# Autodesk Inventor assembly: Miras
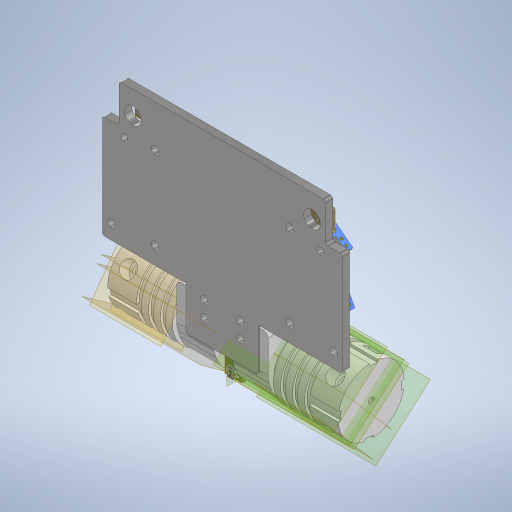
[picture p0: Inventor's stored thumbnail of the model, 512x512]
Saved by Autodesk Inventor 2023.5 (Build 275446000, 446)
## iProperties
Created: 2022-12-28
Part Number: Miras
Document SubType Name: Assembly
Designer: Kamil
Author: Kamil
## Documents named in this file (27)
- E:\PROJECTS_REPOS\Miras\mechanics\Miras.iam
- E:\PROJECTS_REPOS\Miras\mechanics\steel_2.ipt
- E:\PROJECTS_REPOS\Miras\mechanics\lead_3.ipt
- E:\PROJECTS_REPOS\Miras\mechanics\Part8.ipt
- E:\PROJECTS_REPOS\Miras\mechanics\n20 motor.ipt
- E:\PROJECTS_REPOS\Miras\mechanics\felga.ipt
- E:\PROJECTS_REPOS\Miras\mechanics\opona.ipt
- E:\PROJECTS_REPOS\Miras\mechanics\strug.ipt
- E:\PROJECTS_REPOS\Miras\mechanics\sciana.ipt
- E:\PROJECTS_REPOS\Miras\mechanics\sciana_MIR.ipt
- E:\PROJECTS_REPOS\Miras\mechanics\uchwyt na plytke.ipt
- E:\PROJECTS_REPOS\Miras\mechanics\wachlarz_1.ipt
- E:\PROJECTS_REPOS\Miras\mechanics\wachlarz_1_MIR.ipt
- E:\PROJECTS_REPOS\Miras\mechanics\Serwo_z_widelcem.iam
- E:\PROJECTS_REPOS\Miras\mechanics\widelec.ipt
- E:\PROJECTS_REPOS\Miras\mechanics\faulhaber_motor.ipt
- E:\PROJECTS_REPOS\Miras\mechanics\motors_mount_miras.ipt
- E:\PROJECTS_REPOS\Miras\mechanics\wymiar.ipt
- E:\PROJECTS_REPOS\Miras\mechanics\kolo_tetsowe.ipt
- E:\PROJECTS_REPOS\Miras\mechanics\pcb_podstawka.ipt
- E:\PROJECTS_REPOS\Miras\mechanics\plytka_stal_3mm\plytka_stal_3mm.ipt
- E:\PROJECTS_REPOS\Miras\mechanics\pokrywa_stal_3mm\pokrywa_stal_3mm.ipt
- E:\PROJECTS_REPOS\Miras\mechanics\pcb_main_miras v4.ipt
- E:\PROJECTS_REPOS\Miras\mechanics\pcb_top v5.ipt
- E:\PROJECTS_REPOS\Miras\mechanics\Weewooday I2C OLED 0.98_ 128x64.ipt
- C:\Users\kamil\Downloads\Motor\Motor.ipt
- E:\PROJECTS_REPOS\Miras\mechanics\mototrs_Mount_miras_pololu_n20.ipt
## Components (32 placed, 26 different names)
1. steel_2:1 — Mate:4, Mate:5, Flush:1
2. lead_3:1 — Mate:4, Mate:5, Flush:1, Flush:2, Flush:3, Mate:16
3. Part8:1 — Flush:2, Flush:3, Mate:11, Mate:12, Mate:13, Mate:14, Mate:15, Mate:18, Mate:55
4. n20 motor:1 — Mate:10, Mate:11, Mate:13, Mate:14, Mate:19, Mate:20, Mate:21
5. n20 motor:2 — Mate:10, Mate:12, Mate:15, Mate:16, Mate:17, Mate:22
6. felga:1 — Mate:17, Mate:18, Mate:22, Mate:24, Mate:25
7. felga:2 — Mate:19, Mate:20, Mate:21, Mate:23, Mate:26
8. opona:1 — Mate:23, Mate:26, Zestawiające:63
9. opona:2 — Mate:24, Mate:25
10. strug:1 — Mate:29, Mate:31, Zestawiające:68, Równoległe:26, Zestawiające:76, Zestawiające:78
11. sciana:1 — Mate:29, Zestawiające:74, Równoległe:27, Zestawiające:76, Równoległe:28
12. sciana_MIR:1 — Mate:31, Zestawiające:77
13. uchwyt na plytke:1 — Zestawiające:83, Zestawiające:84, Zestawiające:85, Zestawiające:87, Równoległe:30, Zestawiające:88, Zestawiające:89
14. wachlarz_1:2 — Flush:16
15. wachlarz_1_MIR:1 — Flush:16
16. widelec:1 — Mate:55, Mate:56, Mate:57
17. Serwo_z_widelcem:1 [sub-assembly] — Mate:56, Mate:57
18. faulhaber_motor:1 — Kątowe:1, Zestawiające:62, Zestawiające:72
19. faulhaber_motor:2 — Kątowe:1, Zestawiające:62, Zestawiające:63, Zestawiające:71, Zestawiające:73
20. motors_mount_miras:1 — Zestawiające:69, Zestawiające:71, Zestawiające:72, Zestawiające:73, Zestawiające:75, Kątowe:2, Zestawiające:83, Zestawiające:84, Równoległe:30
21. wymiar:1 — Zestawiające:68, Równoległe:26, Zestawiające:69
22. kolo_tetsowe:1 — Zestawiające:91, Zestawiające:93
23. kolo_tetsowe:2 — Zestawiające:90, Zestawiające:92
24. pcb_podstawka:1 — Zestawiające:79, Zestawiające:80, Zestawiające:81, Zestawiające:82
25. plytka_stal_3mm:1 — Zestawiające:74, Równoległe:27, Zestawiające:75, Zestawiające:82, Równoległe:29, Zestawiające:94, Zestawiające:95
26. pokrywa_stal_3mm:1 — Zestawiające:77, Równoległe:28, Zestawiające:78
27. pcb_main_miras v4:1 — Zestawiające:79, Zestawiające:80, Zestawiające:81, Kątowe:2, Równoległe:29, Równoległe:32
28. pcb_top v5:1 — Zestawiające:85
29. Weewooday I2C OLED 0.98_ 128x64:1 — Zestawiające:87, Zestawiające:88, Zestawiające:89
30. Motor:1 — Zestawiające:90, Równoległe:31, Zestawiające:92, Kątowe:3
31. Motor:2 — Zestawiające:91, Równoległe:31, Zestawiające:93
32. mototrs_Mount_miras_pololu_n20:1 — Zestawiające:94, Równoległe:32, Kątowe:3, Zestawiające:95
## Relationships (66: Mate 52, Flush 11, Angle 3)
- Mate:4: steel_2:1 ↔ lead_3:1
- Mate:5: steel_2:1 ↔ lead_3:1
- Flush:1: steel_2:1 ↔ lead_3:1
- Flush:2: lead_3:1 ↔ Part8:1
- Flush:3: lead_3:1 ↔ Part8:1
- Mate:10 (5 mm): n20 motor:1 ↔ n20 motor:2
- Mate:11 (2.5 mm): Part8:1 ↔ n20 motor:1
- Mate:12: Part8:1 ↔ n20 motor:2
- Mate:13: Part8:1 ↔ n20 motor:1
- Mate:14: Part8:1 ↔ n20 motor:1
- Mate:15: Part8:1 ↔ n20 motor:2
- Mate:16: lead_3:1 ↔ n20 motor:2
- Mate:17 (0.5 mm): n20 motor:2 ↔ felga:1
- Mate:18: Part8:1 ↔ felga:1
- Mate:19 (0.5 mm): n20 motor:1 ↔ felga:2
- Mate:20: n20 motor:1 ↔ felga:2
- Mate:21: n20 motor:1 ↔ felga:2
- Mate:22: n20 motor:2 ↔ felga:1
- Mate:23: felga:2 ↔ opona:1
- Mate:24: felga:1 ↔ opona:2
- Mate:25: felga:1 ↔ opona:2
- Mate:26: felga:2 ↔ opona:1
- Mate:29: strug:1 ↔ sciana:1
- Mate:31: strug:1 ↔ sciana_MIR:1
- Flush:16: wachlarz_1:2 ↔ wachlarz_1_MIR:1
- Mate:55: Part8:1 ↔ widelec:1
- Mate:56 (0.5 mm): widelec:1 ↔ Serwo_z_widelcem:1
- Mate:57: widelec:1 ↔ Serwo_z_widelcem:1
- Kątowe:1 [Angle] (180 deg): faulhaber_motor:1 ↔ faulhaber_motor:2
- Zestawiające:62 [Mate]: faulhaber_motor:1 ↔ faulhaber_motor:2
- Zestawiające:63 [Mate]: opona:1 ↔ faulhaber_motor:2
- Zestawiające:68 [Mate]: strug:1 ↔ wymiar:1
- Równoległe:26 [Flush]: strug:1 ↔ wymiar:1
- Zestawiające:69 [Mate] (-50 mm): motors_mount_miras:1 ↔ wymiar:1
- Zestawiające:71 [Mate]: faulhaber_motor:2 ↔ motors_mount_miras:1
- Zestawiające:72 [Mate]: faulhaber_motor:1 ↔ motors_mount_miras:1
- Zestawiające:73 [Mate]: faulhaber_motor:2 ↔ motors_mount_miras:1
- Zestawiające:74 [Mate]: sciana:1 ↔ plytka_stal_3mm:1
- Równoległe:27 [Flush]: sciana:1 ↔ plytka_stal_3mm:1
- Zestawiające:75 [Mate]: motors_mount_miras:1 ↔ plytka_stal_3mm:1
- Zestawiające:76 [Mate]: strug:1 ↔ sciana:1
- Zestawiające:77 [Mate]: sciana_MIR:1 ↔ pokrywa_stal_3mm:1
- Równoległe:28 [Flush]: sciana:1 ↔ pokrywa_stal_3mm:1
- Zestawiające:78 [Mate]: strug:1 ↔ pokrywa_stal_3mm:1
- Zestawiające:79 [Mate]: pcb_podstawka:1 ↔ pcb_main_miras v4:1
- Zestawiające:80 [Mate]: pcb_podstawka:1 ↔ pcb_main_miras v4:1
- Zestawiające:81 [Mate]: pcb_podstawka:1 ↔ pcb_main_miras v4:1
- Zestawiające:82 [Mate]: pcb_podstawka:1 ↔ plytka_stal_3mm:1
- Kątowe:2 [Angle] (0 deg): motors_mount_miras:1 ↔ pcb_main_miras v4:1
- Równoległe:29 [Flush] (-2 mm): plytka_stal_3mm:1 ↔ pcb_main_miras v4:1
- Zestawiające:83 [Mate]: uchwyt na plytke:1 ↔ motors_mount_miras:1
- Zestawiające:84 [Mate]: uchwyt na plytke:1 ↔ motors_mount_miras:1
- Zestawiające:85 [Mate]: uchwyt na plytke:1 ↔ pcb_top v5:1
- Zestawiające:87 [Mate]: uchwyt na plytke:1 ↔ Weewooday I2C OLED 0.98_ 128x64:1
- Równoległe:30 [Flush]: uchwyt na plytke:1 ↔ motors_mount_miras:1
- Zestawiające:88 [Mate]: uchwyt na plytke:1 ↔ Weewooday I2C OLED 0.98_ 128x64:1
- Zestawiające:89 [Mate]: uchwyt na plytke:1 ↔ Weewooday I2C OLED 0.98_ 128x64:1
- Zestawiające:90 [Mate]: kolo_tetsowe:2 ↔ Motor:1
- Zestawiające:91 [Mate]: kolo_tetsowe:1 ↔ Motor:2
- Równoległe:31 [Flush]: Motor:1 ↔ Motor:2
- Zestawiające:92 [Mate] (1 mm): kolo_tetsowe:2 ↔ Motor:1
- Zestawiające:93 [Mate] (1 mm): kolo_tetsowe:1 ↔ Motor:2
- Zestawiające:94 [Mate]: plytka_stal_3mm:1 ↔ mototrs_Mount_miras_pololu_n20:1
- Równoległe:32 [Flush]: pcb_main_miras v4:1 ↔ mototrs_Mount_miras_pololu_n20:1
- Kątowe:3 [Angle] (0 deg): Motor:1 ↔ mototrs_Mount_miras_pololu_n20:1
- Zestawiające:95 [Mate]: plytka_stal_3mm:1 ↔ mototrs_Mount_miras_pololu_n20:1
